# Autodesk Inventor assembly: hips_assembly
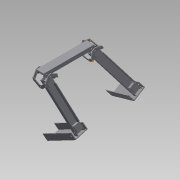
[picture p0: Inventor's stored thumbnail of the model, 180x180]
Saved by Autodesk Inventor 2015 (Build 190159000, 159)
## iProperties
Created: 2014-06-09
Part Number: hips_assembly
Document SubType Name: Assembly
Designer: L
Author: L
## Documents named in this file (3)
- D:\Documents\Autocad\hips_assembly.iam
- D:\Documents\Autocad\upper_leg.iam
- D:\Documents\Autocad\leg_assembly.iam
## Components (3 placed, 2 different names)
1. upper_leg:1 [sub-assembly] — Mate:1, Mate:2, Mate:3, Mate:4, Flush:1, Mate:5
2. leg_assembly:1 [sub-assembly] — Mate:1, Mate:2
3. leg_assembly:2 [sub-assembly] — Mate:3, Mate:4
## Relationships (6: Mate 5, Flush 1)
- Mate:1: upper_leg:1 ↔ leg_assembly:1
- Mate:2: upper_leg:1 ↔ leg_assembly:1
- Mate:3: upper_leg:1 ↔ leg_assembly:2
- Mate:4: upper_leg:1 ↔ leg_assembly:2
- Flush:1: upper_leg:1
- Mate:5: upper_leg:1
